# Autodesk Inventor assembly: Montaje
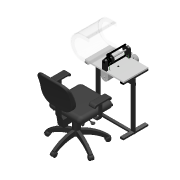
[picture p0: Inventor's stored thumbnail of the model, 180x180]
Saved by Autodesk Inventor 2022 (Build 260153000, 153)
## iProperties
Created: 2019-06-21
Part Number: Montaje
Material: Genérico
Document SubType Name: Assembly
Designer: Cristiano
Author: Cristiano
## Documents named in this file (24)
- G:\Mi unidad\UTEC\Proyectos\Flor de Lana\Diseño 20191119\Montaje.iam
- G:\Mi unidad\UTEC\Proyectos\Flor de Lana\Diseño 20191119\soporte_riel.ipt
- G:\Mi unidad\UTEC\Proyectos\Flor de Lana\Diseño 20191119\soporte_riel2.ipt
- G:\Mi unidad\UTEC\Proyectos\Flor de Lana\Diseño 20191119\DIN 471 - 10x1.ipt
- G:\Mi unidad\UTEC\Proyectos\Flor de Lana\Diseño 20191119\TapaSeguridad\TapaSeguridad.iam
- G:\Mi unidad\UTEC\Proyectos\Flor de Lana\Diseño 20191119\Mesa.iam
- G:\Mi unidad\UTEC\Proyectos\Flor de Lana\Diseño 20191119\TapaEje.iam
- G:\Mi unidad\UTEC\Proyectos\Flor de Lana\Diseño 20191119\TapaEje2.ipt
- G:\Mi unidad\UTEC\Proyectos\Flor de Lana\Diseño 20191119\TapaEje3.ipt
- G:\Mi unidad\UTEC\Proyectos\Flor de Lana\Diseño 20191119\Cadeira_preta.ipt
- C:\Users\cristiano.schuster\Documents\Inventor\Content Center Files\R2022\en-US\ISO 4032(2)\ISO 4032 - M8 - ISO.ipt
- C:\Users\cristiano.schuster\Documents\Inventor\Content Center Files\R2022\en-US\ISO 4014(2)\ISO 4014 - M8 x 55 - ISO.ipt
- C:\Users\cristiano.schuster\Documents\Inventor\Content Center Files\R2022\en-US\ANSI AFBMA 16.1(3)\ANSI_AFBMA 16.1 - 10 x 22 x 6.ipt
- C:\Users\cristiano.schuster\Documents\Inventor\Content Center Files\R2022\en-US\ANSI AFBMA 16.1(1)\ANSI_AFBMA 16.1 - 25 x 47 x 14.ipt
- C:\Users\cristiano.schuster\Documents\Inventor\Content Center Files\R2022\en-US\ISO 4014(2)\ISO 4014 - M10 x 70 - ISO.ipt
- C:\Users\cristiano.schuster\Documents\Inventor\Content Center Files\R2022\en-US\ISO 7089\ISO 7089 - 14 - 140 HV(1).ipt
- C:\Users\cristiano.schuster\Documents\Inventor\Content Center Files\R2022\en-US\ISO 4032(2)\ISO 4032 - M10 - ISO.ipt
- G:\Mi unidad\UTEC\Proyectos\Flor de Lana\Diseño 20191119\Switch.ipt
- G:\Mi unidad\UTEC\Proyectos\Flor de Lana\Diseño 20191119\Montaje Bobinador.iam
- G:\Mi unidad\UTEC\Proyectos\Flor de Lana\Diseño 20191119\Conjunto transimisión.iam
- G:\Mi unidad\UTEC\Proyectos\Flor de Lana\Diseño 20191119\Montaje Reel.iam
- C:\Users\cristiano.schuster\Documents\Inventor\Content Center Files\R2022\en-US\ISO 7045  Z\ISO 7045 - M10 x 60_ - 4.8 - Z - ISO.ipt
- C:\Users\cristiano.schuster\Documents\Inventor\Content Center Files\R2022\en-US\ISO 4035(2)\ISO 4035 - M10 - ISO.ipt
- G:\Mi unidad\UTEC\Proyectos\Flor de Lana\Diseño 20191119\Polea.ipt
## Components (33 placed, 23 different names)
1. soporte_riel:1 — Ángulo:1, Rígido:27, Insert:1, Insert:4, Rotational:33
2. ANSI/AFBMA 16.1 - Airframe Ball Bearings, Single Row, Rigid, Diameter Series 0 25 x 47 x 14:1
3. soporte_riel2:1 — Ángulo:1, Insert:2, Insert:3, Rigid:29, Insert:9, Flush:5, Rotational:36
4. DIN 471 10x1:1 — Rigid:31
5. DIN 471 10x1:2 — Rotational:34
6. Montaje Reel:1 [sub-assembly] — Rotational:35, Rotational:37
7. TapaSeguridad:1 [sub-assembly] — Coincidencia:1, Coincidencia:2, Nivelación:1
8. Mesa:1 [sub-assembly] — Rígido:27, Coincidencia:1, Coincidencia:2, Nivelación:1, Insert:5, Insert:6, Insert:7, Insert:8, Rigid:30, Flush:5, Cylindrical:4, Rigid:36, Rigid:37
9. TapaEje:1 [sub-assembly] — Rigid:34
10. TapaEje3:1 — Rígido:28, Rigid:34
11. TapaEje2:1 — Rígido:28
12. Cadeira_preta:1 — Flush:4
13. ISO 4032 M8:1 — Insert:1
14. ISO 4032 M8:2 — Insert:2
15. ISO 4032 M8:3 — Insert:3
16. ISO 4032 M8:4 — Insert:4
17. ISO 4014 M8 x 55:1 — Insert:5
18. ISO 4014 M8 x 55:2 — Insert:6
19. ISO 4014 M8 x 55:3 — Insert:7
20. ISO 4014 M8 x 55:4 — Insert:8
21. ANSI/AFBMA 16.1 - Airframe Ball Bearings, Single Row, Rigid, Diameter Series 8, 9 10 x 22 x 6:1 — Rigid:29, Cylindrical:3
22. ISO 4014 M10 x 70:1 — Insert:9, Mate:6
23. ISO 7089 14:1 — Mate:7, Rigid:35
24. ISO 4032 M10:1 — Mate:6, Mate:7
25. Switch:1 — Rigid:30
26. Montaje Bobinador:2 [sub-assembly] — Rotational:33, Rigid:31, Rotational:34, Rotational:35, Cylindrical:3, Rigid:38
27. Conjunto transimisión:1 [sub-assembly] — Rotational:36, Cylindrical:4, Rigid:35, Insert:10, Insert:11
28. ISO 7045 Z M10 x 60 - 4.8 - Z:1 — Rigid:36
29. ISO 7045 Z M10 x 60 - 4.8 - Z:2 — Rigid:37
30. ISO 4035 M10:1 — Insert:10
31. ISO 4035 M10:2 — Insert:11
32. Polea:1 — Rigid:38
33. Polea:2 — Rotational:37
## Relationships (37: Insert 11, WeldJoint 10, RevoluteJoint 6, Mate 4, Flush 3, CylindricalJoint 2, Angle 1)
- [RevoluteJoint]: soporte_riel:1 ↔ ANSI/AFBMA 16.1 - Airframe Ball Bearings, Single Row, Rigid, Diameter Series 0 25 x 47 x 14:1
- Ángulo:1 [Angle] (0 deg): soporte_riel:1 ↔ soporte_riel2:1
- Rígido:27 [WeldJoint]: soporte_riel:1 ↔ Mesa:1
- Coincidencia:1 [Mate] (3 mm): TapaSeguridad:1 ↔ Mesa:1
- Coincidencia:2 [Mate] (-110 mm): TapaSeguridad:1 ↔ Mesa:1
- Nivelación:1 [Flush] (-22.5 mm): TapaSeguridad:1 ↔ Mesa:1
- Rígido:28 [WeldJoint]: TapaEje3:1 ↔ TapaEje2:1
- Flush:4 (-350 mm): Cadeira_preta:1
- Insert:1: soporte_riel:1 ↔ ISO 4032 M8:1
- Insert:2: soporte_riel2:1 ↔ ISO 4032 M8:2
- Insert:3: soporte_riel2:1 ↔ ISO 4032 M8:3
- Insert:4: soporte_riel:1 ↔ ISO 4032 M8:4
- Insert:5: Mesa:1 ↔ ISO 4014 M8 x 55:1
- Insert:6: Mesa:1 ↔ ISO 4014 M8 x 55:2
- Insert:7: Mesa:1 ↔ ISO 4014 M8 x 55:3
- Insert:8: Mesa:1 ↔ ISO 4014 M8 x 55:4
- Rigid:29 [WeldJoint]: soporte_riel2:1 ↔ ANSI/AFBMA 16.1 - Airframe Ball Bearings, Single Row, Rigid, Diameter Series 8, 9 10 x 22 x 6:1
- Insert:9: soporte_riel2:1 ↔ ISO 4014 M10 x 70:1
- Mate:6: ISO 4014 M10 x 70:1 ↔ ISO 4032 M10:1
- Mate:7: ISO 7089 14:1 ↔ ISO 4032 M10:1
- Rigid:30 [WeldJoint]: Mesa:1 ↔ Switch:1
- Rotational:33 [RevoluteJoint]: soporte_riel:1 ↔ Montaje Bobinador:2
- Rigid:31 [WeldJoint]: DIN 471 10x1:1 ↔ Montaje Bobinador:2
- Rotational:34 [RevoluteJoint]: DIN 471 10x1:2 ↔ Montaje Bobinador:2
- Rotational:35 [RevoluteJoint]: Montaje Reel:1 ↔ Montaje Bobinador:2
- Cylindrical:3: ANSI/AFBMA 16.1 - Airframe Ball Bearings, Single Row, Rigid, Diameter Series 8, 9 10 x 22 x 6:1 ↔ Montaje Bobinador:2
- Flush:5: soporte_riel2:1 ↔ Mesa:1
- Rigid:34 [WeldJoint] (100 mm): TapaEje:1 ↔ TapaEje3:1
- Rotational:36 [RevoluteJoint]: soporte_riel2:1 ↔ Conjunto transimisión:1
- Cylindrical:4: Mesa:1 ↔ Conjunto transimisión:1
- Rigid:35 [WeldJoint]: ISO 7089 14:1 ↔ Conjunto transimisión:1
- Rigid:36 [WeldJoint]: Mesa:1 ↔ ISO 7045 Z M10 x 60 - 4.8 - Z:1
- Rigid:37 [WeldJoint]: Mesa:1 ↔ ISO 7045 Z M10 x 60 - 4.8 - Z:2
- Insert:10: Conjunto transimisión:1 ↔ ISO 4035 M10:1
- Insert:11: Conjunto transimisión:1 ↔ ISO 4035 M10:2
- Rotational:37 [RevoluteJoint] (2 mm): Montaje Reel:1 ↔ Polea:2
- Rigid:38 [WeldJoint] (-2 mm): Montaje Bobinador:2 ↔ Polea:1
